# Autodesk Inventor assembly: hoop1_cog
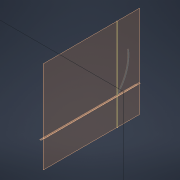
[picture p0: Inventor's stored thumbnail of the model, 180x180]
Saved by Autodesk Inventor 2021 (Build 250183000, 183)
## iProperties
Created: 2021-06-13
Part Number: hoop1_cog
Document SubType Name: Assembly
Designer: Watchdog
Mass: 6071.29 g
Surface Area: 4005.65 cm^2
Volume: 773.413 cm^3
Density: 7.85 g/cm^3
Author: Watchdog
## Documents named in this file (2)
- C:\Users\Watchdog\OneDrive - Flinders\Advn Mech Design Shared\6_Development\2_Design\inventor\hoop_slider\validationfiles\hoop1_cog.iam
- C:\Users\Watchdog\OneDrive - Flinders\Advn Mech Design Shared\6_Development\2_Design\inventor\hoop_slider\large_hoop.ipt
## Components (1 placed, 1 different names)
1. large_hoop:1 — Mate:1, Angle:1, Flush:2, Mate:2
## Relationships (5: Mate 2, Flush 2, Angle 1)
- Mate:1: large_hoop:1
- Angle:1 (0 deg): large_hoop:1
- Flush:1
- Flush:2: large_hoop:1
- Mate:2: large_hoop:1
